# Autodesk Inventor assembly: sorter complete
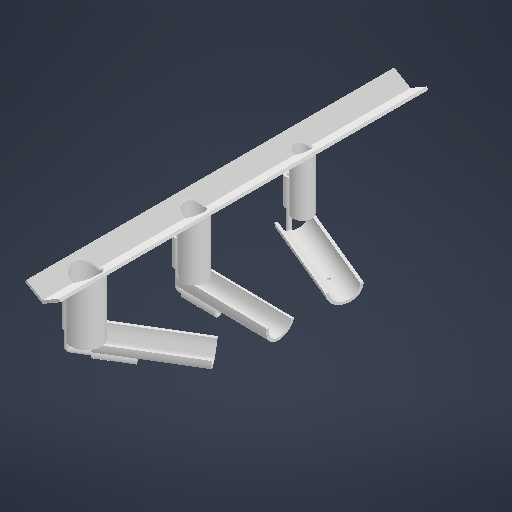
[picture p0: Inventor's stored thumbnail of the model, 512x512]
Saved by Autodesk Inventor 2026.2 (Build 302298010, 298A)
## iProperties
Created: 2026-03-16
Part Number: sorter complete
Document SubType Name: Weldment
Designer: kerel
Weld Material: Welded Aluminum-6061
Author: kerel
## Documents named in this file (4)
- D:\project\sorter complete.iam
- D:\project\sorter.ipt
- D:\project\new part 2 67 kirkified sorter.ipt
- D:\project\new part 3 6767.ipt
## Components (7 placed, 3 different names)
1. sorter:1 — Mate:1, Mate:3, Mate:5
2. new part 2 67 kirkified sorter:1 — Mate:2
3. new part 2 67 kirkified sorter:2 — Mate:4
4. new part 2 67 kirkified sorter:3 — Mate:6
5. new part 3 6767:1 — Mate:1, Mate:2
6. new part 3 6767:2 — Mate:3, Mate:4
7. new part 3 6767:3 — Mate:5, Mate:6
## Relationships (6: Mate 6)
- Mate:1: sorter:1 ↔ new part 3 6767:1
- Mate:2: new part 2 67 kirkified sorter:1 ↔ new part 3 6767:1
- Mate:3: sorter:1 ↔ new part 3 6767:2
- Mate:4: new part 2 67 kirkified sorter:2 ↔ new part 3 6767:2
- Mate:5: sorter:1 ↔ new part 3 6767:3
- Mate:6: new part 2 67 kirkified sorter:3 ↔ new part 3 6767:3
